# Autodesk Inventor assembly: 000 Ensamblaje hw_DAA - BASIC
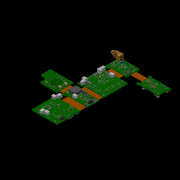
[picture p0: Inventor's stored thumbnail of the model, 180x180]
Saved by Autodesk Inventor 2018 (Build 220112000, 112)
## iProperties
Created: 2024-03-13
Part Number: 000 Ensamblaje hw_DAA - BASIC
Document SubType Name: Assembly
Designer: cda1
Author: cda1
## Documents named in this file (12)
- C:\Users\cda1\Git\DAA\items\hw_DAA\variants\BASIC\3d\En plano\000 Ensamblaje hw_DAA - BASIC.iam
- C:\Users\cda1\Git\DAA\items\hw_DAA\variants\BASIC\3d\000 Ensamblaje hw_DAA - PCB FPGA.iam
- C:\Users\cda1\Git\DAA\items\hw_DAA\variants\BASIC\3d\000 Ensamblaje hw_DAA - PCB Sensor.iam
- C:\Users\cda1\Git\DAA\items\hw_DAA\variants\BASIC\3d\000 Ensamblaje hw_DAA - PCB Lemo.iam
- C:\Users\cda1\Git\DAA\items\hw_DAA\variants\BASIC\3d\000 Ensamblaje hw_DAA - PCB MicroSD.iam
- C:\Users\cda1\Git\DAA\items\hw_DAA\variants\BASIC\3d\000 Ensamblaje hw_DAA - PCB Power.iam
- C:\Users\cda1\Git\DAA\items\hw_DAA\variants\BASIC\3d\000 Ensamblaje hw_DAA - PCB Peripherals.iam
- C:\Users\cda1\Git\DAA\items\hw_DAA\3d\hw_DAA - Flex 1.ipt
- C:\Users\cda1\Git\DAA\items\hw_DAA\3d\hw_DAA - Flex 2.ipt
- C:\Users\cda1\Git\DAA\items\hw_DAA\3d\hw_DAA - Flex 3.ipt
- C:\Users\cda1\Git\DAA\items\hw_DAA\3d\hw_DAA - Flex 4.ipt
- C:\Users\cda1\Git\DAA\items\hw_DAA\3d\hw_DAA - Flex 5.ipt
## Components (11 placed, 11 different names)
1. 000 Ensamblaje hw_DAA - PCB FPGA:1 [sub-assembly] — Coincidencia:5, Ángulo:5, Nivelación:7, Coincidencia:6, Coincidencia:7, Ángulo:6
2. 000 Ensamblaje hw_DAA - PCB Sensor:1 [sub-assembly] — Ángulo:1, Nivelación:1, Coincidencia:4, Ángulo:4, Nivelación:5
3. 000 Ensamblaje hw_DAA - PCB Lemo:1 [sub-assembly] — Nivelación:2
4. 000 Ensamblaje hw_DAA - PCB MicroSD:1 [sub-assembly] — Ángulo:1, Nivelación:1, Nivelación:6
5. 000 Ensamblaje hw_DAA - PCB Power:1 [sub-assembly] — Coincidencia:2, Ángulo:3, Nivelación:4, Coincidencia:3
6. 000 Ensamblaje hw_DAA - PCB Peripherals:1 [sub-assembly] — Coincidencia:1, Ángulo:2, Nivelación:3, Nivelación:8, Coincidencia:8
7. hw_DAA - Flex 1:1 — Coincidencia:1, Ángulo:2, Nivelación:2, Nivelación:3
8. hw_DAA - Flex 2:1 — Coincidencia:2, Ángulo:3, Nivelación:4, Coincidencia:3
9. hw_DAA - Flex 3:1 — Coincidencia:4, Ángulo:4, Nivelación:5, Nivelación:6
10. hw_DAA - Flex 4:1 — Coincidencia:5, Ángulo:5, Nivelación:7, Coincidencia:6
11. hw_DAA - Flex 5:1 — Coincidencia:7, Ángulo:6, Nivelación:8, Coincidencia:8
## Relationships (22: Flush 8, Mate 8, Angle 6)
- Ángulo:1 [Angle] (0 deg): 000 Ensamblaje hw_DAA - PCB Sensor:1 ↔ 000 Ensamblaje hw_DAA - PCB MicroSD:1
- Nivelación:1 [Flush]: 000 Ensamblaje hw_DAA - PCB Sensor:1 ↔ 000 Ensamblaje hw_DAA - PCB MicroSD:1
- Coincidencia:1 [Mate]: 000 Ensamblaje hw_DAA - PCB Peripherals:1 ↔ hw_DAA - Flex 1:1
- Ángulo:2 [Angle] (0 deg): 000 Ensamblaje hw_DAA - PCB Peripherals:1 ↔ hw_DAA - Flex 1:1
- Nivelación:2 [Flush] (7.3 mm): 000 Ensamblaje hw_DAA - PCB Lemo:1 ↔ hw_DAA - Flex 1:1
- Nivelación:3 [Flush] (0.771 mm): 000 Ensamblaje hw_DAA - PCB Peripherals:1 ↔ hw_DAA - Flex 1:1
- Coincidencia:2 [Mate]: 000 Ensamblaje hw_DAA - PCB Power:1 ↔ hw_DAA - Flex 2:1
- Ángulo:3 [Angle] (0 deg): 000 Ensamblaje hw_DAA - PCB Power:1 ↔ hw_DAA - Flex 2:1
- Nivelación:4 [Flush] (0.771 mm): 000 Ensamblaje hw_DAA - PCB Power:1 ↔ hw_DAA - Flex 2:1
- Coincidencia:3 [Mate] (2 mm): 000 Ensamblaje hw_DAA - PCB Power:1 ↔ hw_DAA - Flex 2:1
- Coincidencia:4 [Mate]: 000 Ensamblaje hw_DAA - PCB Sensor:1 ↔ hw_DAA - Flex 3:1
- Ángulo:4 [Angle] (0 deg): 000 Ensamblaje hw_DAA - PCB Sensor:1 ↔ hw_DAA - Flex 3:1
- Nivelación:5 [Flush] (0.771 mm): 000 Ensamblaje hw_DAA - PCB Sensor:1 ↔ hw_DAA - Flex 3:1
- Nivelación:6 [Flush] (7.858 mm): 000 Ensamblaje hw_DAA - PCB MicroSD:1 ↔ hw_DAA - Flex 3:1
- Coincidencia:5 [Mate]: 000 Ensamblaje hw_DAA - PCB FPGA:1 ↔ hw_DAA - Flex 4:1
- Ángulo:5 [Angle] (0 deg): 000 Ensamblaje hw_DAA - PCB FPGA:1 ↔ hw_DAA - Flex 4:1
- Nivelación:7 [Flush] (0.771 mm): 000 Ensamblaje hw_DAA - PCB FPGA:1 ↔ hw_DAA - Flex 4:1
- Coincidencia:6 [Mate] (1.8 mm): 000 Ensamblaje hw_DAA - PCB FPGA:1 ↔ hw_DAA - Flex 4:1
- Coincidencia:7 [Mate]: 000 Ensamblaje hw_DAA - PCB FPGA:1 ↔ hw_DAA - Flex 5:1
- Ángulo:6 [Angle] (0 deg): 000 Ensamblaje hw_DAA - PCB FPGA:1 ↔ hw_DAA - Flex 5:1
- Nivelación:8 [Flush] (0.771 mm): 000 Ensamblaje hw_DAA - PCB Peripherals:1 ↔ hw_DAA - Flex 5:1
- Coincidencia:8 [Mate] (2 mm): 000 Ensamblaje hw_DAA - PCB Peripherals:1 ↔ hw_DAA - Flex 5:1
